# Autodesk Inventor assembly: encoder_ass
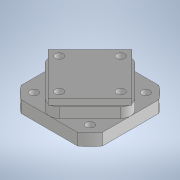
[picture p0: Inventor's stored thumbnail of the model, 180x180]
Saved by Autodesk Inventor 2020 (Build 240168000, 168)
## iProperties
Created: 2019-05-18
Part Number: encoder_ass
Document SubType Name: Assembly
Designer: psrob
Author: psrob
## Documents named in this file (3)
- E:\projects-2\project dog gen2\hardware\encoder_ass.iam
- E:\projects-2\project dog gen2\hardware\encoder_holder.ipt
- E:\projects-2\project dog gen2\hardware\encoder_m.iam
## Components (2 placed, 2 different names)
1. encoder_holder:1 — Insert:1, Insert:2
2. encoder_m:1 [sub-assembly] — Insert:1, Insert:2
## Relationships (2: Insert 2)
- Insert:1: encoder_holder:1 ↔ encoder_m:1
- Insert:2: encoder_holder:1 ↔ encoder_m:1
